# Autodesk Inventor assembly: FP_module
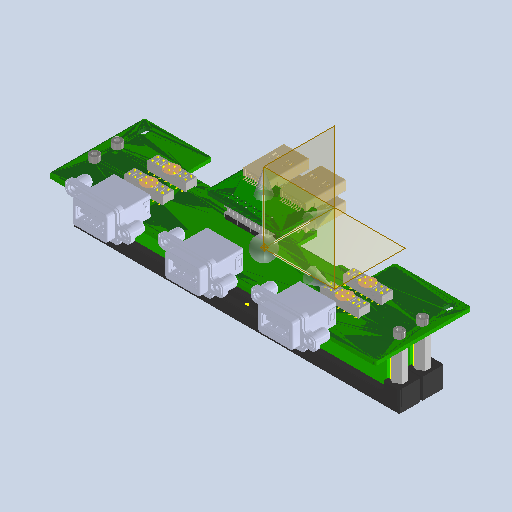
[picture p0: Inventor's stored thumbnail of the model, 512x512]
Saved by Autodesk Inventor 2024.2 (Build 282272000, 272)
## iProperties
Created: 2020-07-14
Part Number: FP_module
Document SubType Name: Assembly
Designer: CASE-SMALL2
Author: CASE-SMALL2
## Documents named in this file (12)
- C:\Users\lgnds\Documents\GitHub\REACH-Hardware\CAD\InventorProject\PCB_Assemblies\FP_module.iam
- C:\Users\lgnds\Documents\GitHub\REACH-Hardware\CAD\InventorProject\PCB_Assemblies\PCB\FP_PCB.ipt
- C:\Users\lgnds\Documents\GitHub\REACH-Hardware\CAD\InventorProject\PCB_Assemblies\Expansion_Module_Assembly.iam
- C:\Users\lgnds\Documents\GitHub\REACH-Hardware\CAD\InventorProject\PCB_Assemblies\Connector\HLE-107-02-F-DV-BE-A\HLE-107-02-F-DV-BE-A.iam
- C:\Users\lgnds\Documents\GitHub\REACH-Hardware\CAD\InventorProject\PCB_Assemblies\PCB\FP_USB_PCB.ipt
- C:\Users\lgnds\Documents\GitHub\REACH-Hardware\CAD\InventorProject\PCB_Assemblies\Connector\TW-10-11-T-D-250-080\TW-10-11-T-D-250-080.iam
- C:\Users\lgnds\Documents\GitHub\REACH-Hardware\CAD\InventorProject\PCB_Assemblies\Connector\GSB3164X1CEU.ipt
- C:\Users\lgnds\Documents\GitHub\REACH-Hardware\CAD\InventorProject\PCB_Assemblies\Screws\ISO 4762 - M2.5 x 5ISO.ipt
- C:\Users\lgnds\Documents\GitHub\REACH-Hardware\CAD\InventorProject\PCB_Assemblies\Screws\DIN 125 - A 2.8.ipt
- C:\Users\lgnds\Documents\GitHub\REACH-Hardware\CAD\InventorProject\PCB_Assemblies\Screws\ISO 4762 - M2.5 x 8ISO.ipt
- C:\Users\lgnds\Documents\GitHub\REACH-Hardware\CAD\InventorProject\PCB_Assemblies\PCBA_Models\FP-PCBA-R2\FP-PCBA-R2.iam
- C:\Users\lgnds\Documents\GitHub\REACH-Hardware\CAD\InventorProject\PCB_Assemblies\PCBA_Models\USB-EXT\USB-EXT.iam
## Components (27 placed, 11 different names)
1. FP_PCB:1 — Rigid:1, Rigid:2, Mate:1, Mate:2, Mate:3, Mate:4, Flush:3, Flush:5, Flush:7, Flush:8, Mate:5, Flush:11, Flush:12, Mate:9, Mate:10, Mate:11, Mate:12, Flush:13, Rigid:3, Rigid:4, Rigid:5, Rigid:6, Rigid:11
2. FP-PCBA-R2:1 [sub-assembly] — Rigid:11
3. Expansion_Module_Assembly:1 [sub-assembly] — Rigid:1, Rotational:1, Rotational:3
4. Expansion_Module_Assembly:2 [sub-assembly] — Rigid:2, Rotational:2, Rotational:4
5. HLE-107-02-F-DV-BE-A:1 [sub-assembly] — Mate:2, Flush:2, Flush:4, Flush:5
6. HLE-107-02-F-DV-BE-A:2 [sub-assembly] — Mate:1, Flush:2, Flush:3, Flush:4
7. HLE-107-02-F-DV-BE-A:3 [sub-assembly] — Mate:3, Flush:1, Flush:6, Flush:7, Flush:8
8. HLE-107-02-F-DV-BE-A:4 [sub-assembly] — Mate:4, Flush:1, Flush:6
9. FP_USB_PCB:1 — Mate:5, Flush:11, Flush:12, Mate:7, Mate:8, Mate:13, Mate:14, Mate:17, Mate:19, Mate:20, Mate:21, Rigid:12
10. USB-EXT:1 [sub-assembly] — Rigid:12
11. TW-10-11-T-D-250-080:1 [sub-assembly] — Flush:13, Mate:19, Mate:20
12. GSB3164X1CEU:1 — Mate:7, Mate:14, Mate:15, Mate:17
13. GSB3164X1CEU:2 — Mate:8, Mate:13, Mate:15
14. GSB3164X1CEU:3 — Mate:9, Mate:12, Mate:16
15. GSB3164X1CEU:4 — Mate:10, Mate:11, Mate:16, Mate:21
16. ISO 4762 - M2.5 x 5ISO:1 — Rigid:4
17. ISO 4762 - M2.5 x 5ISO:2 — Rigid:3
18. ISO 4762 - M2.5 x 5ISO:3 — Rigid:6
19. ISO 4762 - M2.5 x 5ISO:4 — Rigid:5
20. DIN 125 - A 2.8:1 — Rotational:1, Rigid:8
21. DIN 125 - A 2.8:2 — Rotational:2, Rigid:7
22. DIN 125 - A 2.8:3 — Rotational:3, Rigid:10
23. DIN 125 - A 2.8:4 — Rotational:4, Rigid:9
24. ISO 4762 - M2.5 x 8ISO:1 — Rigid:9
25. ISO 4762 - M2.5 x 8ISO:2 — Rigid:10
26. ISO 4762 - M2.5 x 8ISO:3 — Rigid:8
27. ISO 4762 - M2.5 x 8ISO:4 — Rigid:7
## Relationships (46: Mate 19, WeldJoint 12, Flush 11, RevoluteJoint 4)
- Rigid:1 [WeldJoint]: FP_PCB:1 ↔ Expansion_Module_Assembly:1
- Rigid:2 [WeldJoint]: FP_PCB:1 ↔ Expansion_Module_Assembly:2
- Mate:1: FP_PCB:1 ↔ HLE-107-02-F-DV-BE-A:2
- Mate:2: FP_PCB:1 ↔ HLE-107-02-F-DV-BE-A:1
- Mate:3: FP_PCB:1 ↔ HLE-107-02-F-DV-BE-A:3
- Mate:4: FP_PCB:1 ↔ HLE-107-02-F-DV-BE-A:4
- Flush:1 (10.5 mm): HLE-107-02-F-DV-BE-A:3 ↔ HLE-107-02-F-DV-BE-A:4
- Flush:2 (10.5 mm): HLE-107-02-F-DV-BE-A:1 ↔ HLE-107-02-F-DV-BE-A:2
- Flush:3 (14.96 mm): FP_PCB:1 ↔ HLE-107-02-F-DV-BE-A:2
- Flush:4: HLE-107-02-F-DV-BE-A:1 ↔ HLE-107-02-F-DV-BE-A:2
- Flush:5 (21.11 mm): FP_PCB:1 ↔ HLE-107-02-F-DV-BE-A:1
- Flush:6: HLE-107-02-F-DV-BE-A:3 ↔ HLE-107-02-F-DV-BE-A:4
- Flush:7 (14.96 mm): FP_PCB:1 ↔ HLE-107-02-F-DV-BE-A:3
- Flush:8 (21.11 mm): FP_PCB:1 ↔ HLE-107-02-F-DV-BE-A:3
- Mate:5 (6.9 mm): FP_PCB:1 ↔ FP_USB_PCB:1
- Flush:11: FP_PCB:1 ↔ FP_USB_PCB:1
- Flush:12 (68.1 mm): FP_PCB:1 ↔ FP_USB_PCB:1
- Mate:7 (0.5 mm): FP_USB_PCB:1 ↔ GSB3164X1CEU:1
- Mate:8 (0.5 mm): FP_USB_PCB:1 ↔ GSB3164X1CEU:2
- Mate:9 (0.5 mm): FP_PCB:1 ↔ GSB3164X1CEU:3
- Mate:10 (0.5 mm): FP_PCB:1 ↔ GSB3164X1CEU:4
- Mate:11: FP_PCB:1 ↔ GSB3164X1CEU:4
- Mate:12: FP_PCB:1 ↔ GSB3164X1CEU:3
- Mate:13: FP_USB_PCB:1 ↔ GSB3164X1CEU:2
- Mate:14: FP_USB_PCB:1 ↔ GSB3164X1CEU:1
- Mate:15 (5 mm): GSB3164X1CEU:1 ↔ GSB3164X1CEU:2
- Mate:16 (5 mm): GSB3164X1CEU:3 ↔ GSB3164X1CEU:4
- Mate:17 (2.5 mm): FP_USB_PCB:1 ↔ GSB3164X1CEU:1
- Flush:13 (12.502 mm): FP_PCB:1 ↔ TW-10-11-T-D-250-080:1
- Mate:19 (0.1 mm): FP_USB_PCB:1 ↔ TW-10-11-T-D-250-080:1
- Mate:20: FP_USB_PCB:1 ↔ TW-10-11-T-D-250-080:1
- Mate:21 (2.5 mm): FP_USB_PCB:1 ↔ GSB3164X1CEU:4
- Rigid:3 [WeldJoint]: FP_PCB:1 ↔ ISO 4762 - M2.5 x 5ISO:2
- Rigid:4 [WeldJoint]: FP_PCB:1 ↔ ISO 4762 - M2.5 x 5ISO:1
- Rigid:5 [WeldJoint]: FP_PCB:1 ↔ ISO 4762 - M2.5 x 5ISO:4
- Rigid:6 [WeldJoint]: FP_PCB:1 ↔ ISO 4762 - M2.5 x 5ISO:3
- Rotational:1 [RevoluteJoint]: Expansion_Module_Assembly:1 ↔ DIN 125 - A 2.8:1
- Rotational:2 [RevoluteJoint]: Expansion_Module_Assembly:2 ↔ DIN 125 - A 2.8:2
- Rotational:3 [RevoluteJoint]: Expansion_Module_Assembly:1 ↔ DIN 125 - A 2.8:3
- Rotational:4 [RevoluteJoint]: Expansion_Module_Assembly:2 ↔ DIN 125 - A 2.8:4
- Rigid:7 [WeldJoint]: DIN 125 - A 2.8:2 ↔ ISO 4762 - M2.5 x 8ISO:4
- Rigid:8 [WeldJoint]: DIN 125 - A 2.8:1 ↔ ISO 4762 - M2.5 x 8ISO:3
- Rigid:9 [WeldJoint]: DIN 125 - A 2.8:4 ↔ ISO 4762 - M2.5 x 8ISO:1
- Rigid:10 [WeldJoint]: DIN 125 - A 2.8:3 ↔ ISO 4762 - M2.5 x 8ISO:2
- Rigid:11 [WeldJoint]: FP_PCB:1 ↔ FP-PCBA-R2:1
- Rigid:12 [WeldJoint]: FP_USB_PCB:1 ↔ USB-EXT:1
